# Autodesk Inventor assembly: mg996r_right_top_rot_frame
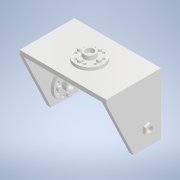
[picture p0: Inventor's stored thumbnail of the model, 180x180]
Saved by Autodesk Inventor 2021.4 (Build 254397000, 397)
## iProperties
Created: 2022-07-25
Part Number: mg996r_right_top_rot_frame
Document SubType Name: Assembly
Designer: isamu
Author: isamu
## Documents named in this file (6)
- D:\personal_projects\robot\inventor\2021_matlab_compat\mg996r_right_top_rot_frame.iam
- D:\personal_projects\robot\exports\frames\servo frame mg996 centered_MIR.ipt
- D:\personal_projects\robot\exports\handle\servo handle 4.ipt
- D:\personal_projects\robot\exports\screws\m2 nuts.ipt
- D:\personal_projects\robot\exports\screws\m2x8.ipt
- D:\personal_projects\robot\exports\screws\m4 nuts.ipt
## Components (20 placed, 5 different names)
1. servo frame mg996 centered_MIR:1 — Insert:1, Mate:1, Mate:2, Mate:3, Mate:4, Mate:5, Mate:6, Insert:6, Insert:7, Insert:8, Insert:9, Insert:14, Insert:15, Insert:16, Insert:17
2. servo handle 4:1 — Mate:1, Mate:2, Mate:3, Insert:2, Insert:3, Insert:4, Insert:5
3. servo handle 4:2 — Mate:4, Mate:5, Mate:6, Insert:10, Insert:11, Insert:12, Insert:13
4. m2 nuts:1 — Insert:7
5. m2 nuts:2 — Insert:6
6. m2 nuts:3 — Insert:8
7. m2 nuts:4 — Insert:14
8. m2 nuts:5 — Insert:9
9. m2 nuts:6 — Insert:15
10. m2 nuts:7 — Insert:16
11. m2 nuts:8 — Insert:17
12. m2x8:1 — Insert:11
13. m2x8:2 — Insert:5
14. m2x8:3 — Insert:12
15. m2x8:4 — Insert:13
16. m2x8:5 — Insert:2
17. m2x8:6 — Insert:3
18. m2x8:7 — Insert:4
19. m2x8:8 — Insert:10
20. m4 nuts:1 — Insert:1
## Relationships (23: Insert 17, Mate 6)
- Insert:1: servo frame mg996 centered_MIR:1 ↔ m4 nuts:1
- Mate:1: servo frame mg996 centered_MIR:1 ↔ servo handle 4:1
- Mate:2: servo frame mg996 centered_MIR:1 ↔ servo handle 4:1
- Mate:3: servo frame mg996 centered_MIR:1 ↔ servo handle 4:1
- Mate:4: servo frame mg996 centered_MIR:1 ↔ servo handle 4:2
- Mate:5: servo frame mg996 centered_MIR:1 ↔ servo handle 4:2
- Mate:6: servo frame mg996 centered_MIR:1 ↔ servo handle 4:2
- Insert:2: servo handle 4:1 ↔ m2x8:5
- Insert:3: servo handle 4:1 ↔ m2x8:6
- Insert:4: servo handle 4:1 ↔ m2x8:7
- Insert:5: servo handle 4:1 ↔ m2x8:2
- Insert:6: servo frame mg996 centered_MIR:1 ↔ m2 nuts:2
- Insert:7: servo frame mg996 centered_MIR:1 ↔ m2 nuts:1
- Insert:8: servo frame mg996 centered_MIR:1 ↔ m2 nuts:3
- Insert:9: servo frame mg996 centered_MIR:1 ↔ m2 nuts:5
- Insert:10: servo handle 4:2 ↔ m2x8:8
- Insert:11: servo handle 4:2 ↔ m2x8:1
- Insert:12: servo handle 4:2 ↔ m2x8:3
- Insert:13: servo handle 4:2 ↔ m2x8:4
- Insert:14: servo frame mg996 centered_MIR:1 ↔ m2 nuts:4
- Insert:15: servo frame mg996 centered_MIR:1 ↔ m2 nuts:6
- Insert:16: servo frame mg996 centered_MIR:1 ↔ m2 nuts:7
- Insert:17: servo frame mg996 centered_MIR:1 ↔ m2 nuts:8
